# Autodesk Inventor assembly: CAD_Assembly
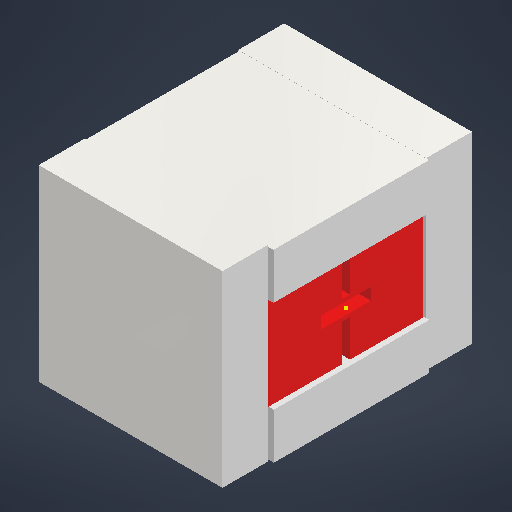
[picture p0: Inventor's stored thumbnail of the model, 512x512]
Saved by Autodesk Inventor 2026.2 (Build 302298000, 298)
## iProperties
Created: 2026-07-02
Part Number: CAD_Assembly
Document SubType Name: Assembly
Designer: usman
Author: usman
## Documents named in this file (6)
- C:\Users\usman\OneDrive - Georgia Southern University\Desktop\USC-1stSemester\NMR\Compact-NMR\System_development\magnet_design\A650-290\CAD\CAD_Assembly.iam
- C:\Users\usman\OneDrive - Georgia Southern University\Desktop\USC-1stSemester\NMR\Compact-NMR\System_development\magnet_design\A650-290\CAD\Concave_3_516_Plate.ipt
- C:\Users\usman\OneDrive - Georgia Southern University\Desktop\USC-1stSemester\NMR\Compact-NMR\System_development\magnet_design\A650-290\CAD\Metal_Bar1.ipt
- C:\Users\usman\OneDrive - Georgia Southern University\Desktop\USC-1stSemester\NMR\Compact-NMR\System_development\magnet_design\A650-290\CAD\Metal_Bar2.ipt
- C:\Users\usman\OneDrive - Georgia Southern University\Desktop\USC-1stSemester\NMR\Compact-NMR\System_development\magnet_design\A650-290\CAD\SampleMagnet.ipt
- C:\Users\usman\OneDrive - Georgia Southern University\Desktop\USC-1stSemester\NMR\Compact-NMR\System_development\magnet_design\A650-290\CAD\Base_Casing_A0645.ipt
## Components (9 placed, 5 different names)
1. Concave_3_516_Plate:1 — Rigid:1, Rigid:2
2. Metal_Bar1:1 — Rigid:6, Flush:2
3. Metal_Bar2:1 — Rigid:4, Flush:1, Flush:2
4. SampleMagnet:1 — Rigid:2, Rigid:6
5. Base_Casing_A0645:1 — Rigid:1, Rigid:3, Rigid:4, Rigid:5
6. Concave_3_516_Plate:2 — Rigid:3, Rotational:1
7. Metal_Bar1:2 — Rigid:7, Flush:1
8. Metal_Bar2:2 — Rigid:5
9. SampleMagnet:2 — Rotational:1, Rigid:7
## Relationships (10: WeldJoint 7, Flush 2, RevoluteJoint 1)
- Rigid:1 [WeldJoint]: Concave_3_516_Plate:1 ↔ Base_Casing_A0645:1
- Rigid:2 [WeldJoint]: Concave_3_516_Plate:1 ↔ SampleMagnet:1
- Rigid:3 [WeldJoint]: Base_Casing_A0645:1 ↔ Concave_3_516_Plate:2
- Rotational:1 [RevoluteJoint]: Concave_3_516_Plate:2 ↔ SampleMagnet:2
- Rigid:4 [WeldJoint]: Metal_Bar2:1 ↔ Base_Casing_A0645:1
- Rigid:5 [WeldJoint]: Base_Casing_A0645:1 ↔ Metal_Bar2:2
- Rigid:6 [WeldJoint]: Metal_Bar1:1 ↔ SampleMagnet:1
- Rigid:7 [WeldJoint]: Metal_Bar1:2 ↔ SampleMagnet:2
- Flush:1: Metal_Bar2:1 ↔ Metal_Bar1:2
- Flush:2: Metal_Bar1:1 ↔ Metal_Bar2:1
## Named parameters: Finish1_Area = 1218.03, Finish2_Area = 38.0031, Finish3_Area = 215.76, Finish4_Area = 215.76, Finish5_Area = 773.249
note: some values were not read from the file. Shown as the stored number, unit unknown: "Finish1_Area", "Finish2_Area", "Finish3_Area", "Finish4_Area", "Finish5_Area".
